# Autodesk Inventor assembly: LaundryRobot_v01
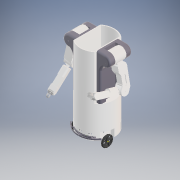
[picture p0: Inventor's stored thumbnail of the model, 180x180]
Saved by Autodesk Inventor 2017 SP1 (Build 210196100, 196)
## iProperties
Created: 2017-03-11
Part Number: LaundryRobot_v01
Document SubType Name: Assembly
Designer: zallen
Author: zallen
## Documents named in this file (3)
- C:\Users\Zach\Documents\Autodesk Inventor Projects\LaundryRobot_v0.1\LaundryRobot_v01.iam
- C:\Users\Zach\Documents\Autodesk Inventor Projects\LaundryRobot_v0.1\Base\Base.iam
- C:\Users\Zach\Documents\Autodesk Inventor Projects\LaundryRobot_v0.1\Body\Body.iam
## Components (2 placed, 2 different names)
1. Base:1 [sub-assembly] — Mate:1, Mate:2
2. Body:1 [sub-assembly] — Mate:1, Mate:2
## Relationships (2: Mate 2)
- Mate:1: Base:1 ↔ Body:1
- Mate:2: Base:1 ↔ Body:1
